# Autodesk Inventor assembly: OpticsTable_Shelf
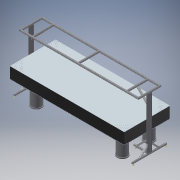
[picture p0: Inventor's stored thumbnail of the model, 180x180]
Saved by Autodesk Inventor 2018 (Build 220112000, 112)
## iProperties
Created: 2018-01-27
Part Number: OpticsTable_Shelf
Document SubType Name: Assembly
Designer: Rich
Author: Rich
## Documents named in this file (14)
- C:\Users\Rich\development\UWaterloo\opticstable_shelf\OpticsTable_Shelf.iam
- C:\Users\Rich\development\UWaterloo\opticstable_shelf\8020-1515-LS-1515-LS X 310cm.ipt
- C:\Users\Rich\development\UWaterloo\opticstable_shelf\8020-1545-S-1545-S X 54.ipt
- C:\Users\Rich\development\UWaterloo\opticstable_shelf\8020-1515-LS-1515-LS X 24.ipt
- C:\Users\Rich\development\UWaterloo\opticstable_shelf\8020-1515-LS-1515-LS X 21.ipt
- C:\Users\Rich\development\UWaterloo\opticstable_shelf\8020 Original Parts\8020-3660-DEFAULT.ipt
- C:\Users\Rich\development\UWaterloo\opticstable_shelf\8020-1515-LS-1515-LS X 36.ipt
- C:\Users\Rich\development\UWaterloo\opticstable_shelf\8020 Original Parts\8020-2561-$PARTNUMBER.ipt
- C:\Users\Rich\development\UWaterloo\opticstable_shelf\8020 Original Parts\8020-2563-$PARTNUMBER.ipt
- C:\Users\Rich\development\UWaterloo\opticstable_shelf\8020 Original Parts\8020-2190-DEFAULT.ipt
- C:\Users\Rich\development\UWaterloo\opticstable_shelf\8020 Original Parts\8020-2200-DEFAULT.ipt
- C:\Users\Rich\development\UWaterloo\opticstable_shelf\8020-1515-S-1515-S X 15.ipt
- C:\Users\Rich\development\UWaterloo\opticstable_shelf\8020 Original Parts\RS2000-410-12.ipt
- C:\Users\Rich\development\UWaterloo\opticstable_shelf\8020 Original Parts\Newport SL 1200-422.ipt
## Components (53 placed, 13 different names)
1. 8020-1545-S-1545-S X 54:1 — Flush:14, Mate:8, Mate:12, Flush:21, Flush:22, Flush:26, Mate:18, Mate:25, Flush:29, Mate:26, Flush:33, Flush:37, Mate:32, Angle:6, Flush:38, Mate:33, Angle:7, Flush:41, Mate:36, Angle:10, Flush:42, Mate:37, Angle:11, Mate:50, Flush:53
2. 8020-1515-LS-1515-LS X 310cm:1 — Mate:3, Flush:5, Flush:6, Flush:11, Mate:6, Flush:12, Mate:9, Flush:15, Mate:10, Flush:16, Flush:24, Mate:13, Flush:25, Mate:14, Angle:1
3. 8020-1515-LS-1515-LS X 310cm:2 — Mate:4, Flush:7, Flush:8, Mate:5, Flush:9, Flush:10, Flush:17, Mate:11, Flush:31, Mate:28, Angle:2, Flush:32, Mate:29, Angle:3
4. 8020-1545-S-1545-S X 54:2 — Mate:2, Flush:4, Mate:7, Flush:13, Flush:18, Flush:20, Flush:21, Mate:15, Mate:16, Mate:21, Flush:27, Mate:23, Flush:34, Mate:30, Flush:35, Angle:4, Mate:31, Flush:36, Angle:5, Flush:39, Mate:34, Angle:8, Flush:40, Mate:35, Angle:9, Mate:49, Flush:52
5. 8020-1515-LS-1515-LS X 24:1 — Mate:5, Flush:9, Flush:10, Flush:11, Mate:6, Flush:12, Flush:14, Mate:8
6. 8020-1515-LS-1515-LS X 24:2 — Mate:3, Flush:5, Flush:6, Mate:4, Flush:7, Flush:8, Mate:7, Flush:13, Flush:20, Flush:23
7. 8020-1515-LS-1515-LS X 21:1 — Mate:9, Flush:15, Mate:17, Mate:46, Flush:51, Angle:16, Mate:47, Mate:48, Angle:17
8. 8020-1515-LS-1515-LS X 21:2 — Mate:10, Flush:16, Flush:23, Mate:44, Flush:49, Angle:14, Mate:45, Flush:50, Angle:15
9. 8020-1515-LS-1515-LS X 21:3 — Flush:17, Mate:11, Mate:19, Flush:47, Mate:42, Angle:12, Flush:48, Mate:43, Angle:13
10. 8020-1515-LS-1515-LS X 36:1 — Mate:12, Flush:19, Flush:22, Mate:24, Mate:27, Flush:30, Mate:38, Flush:43, Mate:39, Flush:44, Mate:51, Flush:54
11. 8020-1515-LS-1515-LS X 36:2 — Mate:1, Mate:2, Flush:4, Flush:18, Flush:19, Mate:20, Mate:22, Flush:28, Mate:40, Flush:45, Mate:41, Flush:46, Mate:52, Flush:56
12. 8020-3660-DEFAULT:1 — Flush:24, Mate:13, Angle:1
13. 8020-3660-DEFAULT:2 — Flush:25, Mate:14
14. 8020-2561-$PARTNUMBER:1 — Mate:22, Mate:23, Flush:28
15. 8020-2561-$PARTNUMBER:2 — Mate:24, Mate:25, Flush:29
16. 8020-2563-$PARTNUMBER:1 — Mate:16, Mate:17, Flush:34
17. 8020-2563-$PARTNUMBER:2 — Mate:18, Mate:19, Flush:33
18. 8020-2561-$PARTNUMBER:3 — Mate:26, Mate:27, Flush:30
19. 8020-2561-$PARTNUMBER:4 — Mate:20, Mate:21, Flush:27
20. 8020-2190-DEFAULT:1
21. 8020-2190-DEFAULT:2
22. 8020-2190-DEFAULT:3
23. 8020-3660-DEFAULT:3 — Flush:31, Mate:28, Angle:2
24. 8020-3660-DEFAULT:4 — Flush:32, Mate:29, Angle:3
25. 8020-3660-DEFAULT:5 — Mate:30, Flush:35, Angle:4
26. 8020-3660-DEFAULT:6 — Mate:31, Flush:36, Angle:5
27. 8020-3660-DEFAULT:7 — Flush:37, Mate:32, Angle:6
28. 8020-3660-DEFAULT:8 — Flush:38, Mate:33, Angle:7
29. 8020-3660-DEFAULT:9 — Flush:39, Mate:34, Angle:8
30. 8020-3660-DEFAULT:10 — Flush:40, Mate:35, Angle:9
31. 8020-3660-DEFAULT:11 — Flush:41, Mate:36, Angle:10
32. 8020-3660-DEFAULT:12 — Flush:42, Mate:37, Angle:11
33. 8020-2200-DEFAULT:1 — Mate:38, Flush:43
34. 8020-2200-DEFAULT:2 — Mate:39, Flush:44
35. 8020-2200-DEFAULT:3 — Mate:40, Flush:45
36. 8020-2200-DEFAULT:4 — Mate:41, Flush:46
37. 8020-3660-DEFAULT:13 — Flush:47, Mate:42, Angle:12
38. 8020-3660-DEFAULT:14 — Flush:48, Mate:43, Angle:13
39. 8020-3660-DEFAULT:15 — Mate:44, Flush:49, Angle:14
40. 8020-3660-DEFAULT:16 — Mate:45, Flush:50, Angle:15
41. 8020-3660-DEFAULT:17 — Mate:46, Flush:51, Angle:16
42. 8020-3660-DEFAULT:18 — Mate:47, Mate:48, Angle:17
43. 8020-2563-$PARTNUMBER:3 — Mate:49, Flush:52, Flush:57, Mate:53
44. 8020-2563-$PARTNUMBER:4 — Mate:50, Flush:53, Flush:55, Mate:54
45. 8020-1515-S-1515-S X 15:1 — Mate:51, Flush:54, Flush:55, Mate:54, Mate:56, Flush:59
46. 8020-1515-S-1515-S X 15:2 — Mate:52, Flush:56, Flush:57, Mate:53, Mate:55, Flush:58
47. 8020-2200-DEFAULT:5 — Mate:55, Flush:58
48. 8020-2200-DEFAULT:6 — Mate:56, Flush:59
49. RS2000-410-12:1 — Mate:57, Mate:58, Flush:60
50. Newport SL 1200-422:1 — Mate:57, Mate:58, Flush:60, Mate:59
51. Newport SL 1200-422:2
52. Newport SL 1200-422:3
53. Newport SL 1200-422:4
## Component patterns: (4 elements, first: Newport SL 1200-422:1)
## Relationships (133: Mate 59, Flush 57, Angle 17)
- Mate:1: 8020-1515-LS-1515-LS X 36:2
- Mate:2: 8020-1545-S-1545-S X 54:2 ↔ 8020-1515-LS-1515-LS X 36:2
- Flush:4: 8020-1545-S-1545-S X 54:2 ↔ 8020-1515-LS-1515-LS X 36:2
- Mate:3: 8020-1515-LS-1515-LS X 310cm:1 ↔ 8020-1515-LS-1515-LS X 24:2
- Flush:5: 8020-1515-LS-1515-LS X 310cm:1 ↔ 8020-1515-LS-1515-LS X 24:2
- Flush:6: 8020-1515-LS-1515-LS X 310cm:1 ↔ 8020-1515-LS-1515-LS X 24:2
- Mate:4: 8020-1515-LS-1515-LS X 310cm:2 ↔ 8020-1515-LS-1515-LS X 24:2
- Flush:7: 8020-1515-LS-1515-LS X 310cm:2 ↔ 8020-1515-LS-1515-LS X 24:2
- Flush:8: 8020-1515-LS-1515-LS X 310cm:2 ↔ 8020-1515-LS-1515-LS X 24:2
- Mate:5: 8020-1515-LS-1515-LS X 310cm:2 ↔ 8020-1515-LS-1515-LS X 24:1
- Flush:9: 8020-1515-LS-1515-LS X 310cm:2 ↔ 8020-1515-LS-1515-LS X 24:1
- Flush:10: 8020-1515-LS-1515-LS X 310cm:2 ↔ 8020-1515-LS-1515-LS X 24:1
- Flush:11: 8020-1515-LS-1515-LS X 310cm:1 ↔ 8020-1515-LS-1515-LS X 24:1
- Mate:6: 8020-1515-LS-1515-LS X 310cm:1 ↔ 8020-1515-LS-1515-LS X 24:1
- Flush:12: 8020-1515-LS-1515-LS X 310cm:1 ↔ 8020-1515-LS-1515-LS X 24:1
- Mate:7: 8020-1545-S-1545-S X 54:2 ↔ 8020-1515-LS-1515-LS X 24:2
- Flush:13: 8020-1545-S-1545-S X 54:2 ↔ 8020-1515-LS-1515-LS X 24:2
- Flush:14: 8020-1545-S-1545-S X 54:1 ↔ 8020-1515-LS-1515-LS X 24:1
- Mate:8: 8020-1545-S-1545-S X 54:1 ↔ 8020-1515-LS-1515-LS X 24:1
- Mate:9: 8020-1515-LS-1515-LS X 310cm:1 ↔ 8020-1515-LS-1515-LS X 21:1
- Flush:15: 8020-1515-LS-1515-LS X 310cm:1 ↔ 8020-1515-LS-1515-LS X 21:1
- Mate:10: 8020-1515-LS-1515-LS X 310cm:1 ↔ 8020-1515-LS-1515-LS X 21:2
- Flush:16: 8020-1515-LS-1515-LS X 310cm:1 ↔ 8020-1515-LS-1515-LS X 21:2
- Flush:17: 8020-1515-LS-1515-LS X 310cm:2 ↔ 8020-1515-LS-1515-LS X 21:3
- Mate:11: 8020-1515-LS-1515-LS X 310cm:2 ↔ 8020-1515-LS-1515-LS X 21:3
- Mate:12: 8020-1545-S-1545-S X 54:1 ↔ 8020-1515-LS-1515-LS X 36:1
- Flush:18 (-400.05 mm): 8020-1545-S-1545-S X 54:2 ↔ 8020-1515-LS-1515-LS X 36:2
- Flush:19: 8020-1515-LS-1515-LS X 36:1 ↔ 8020-1515-LS-1515-LS X 36:2
- Flush:20 (247.65 mm): 8020-1545-S-1545-S X 54:2 ↔ 8020-1515-LS-1515-LS X 24:2
- Flush:21: 8020-1545-S-1545-S X 54:1 ↔ 8020-1545-S-1545-S X 54:2
- Flush:22: 8020-1545-S-1545-S X 54:1 ↔ 8020-1515-LS-1515-LS X 36:1
- Flush:23 (-1530.95 mm): 8020-1515-LS-1515-LS X 24:2 ↔ 8020-1515-LS-1515-LS X 21:2
- Flush:24: 8020-1515-LS-1515-LS X 310cm:1 ↔ 8020-3660-DEFAULT:1
- Mate:13: 8020-1515-LS-1515-LS X 310cm:1 ↔ 8020-3660-DEFAULT:1
- Flush:25: 8020-1515-LS-1515-LS X 310cm:1 ↔ 8020-3660-DEFAULT:2
- Mate:14: 8020-1515-LS-1515-LS X 310cm:1 ↔ 8020-3660-DEFAULT:2
- Flush:26: 8020-1545-S-1545-S X 54:1
- Angle:1 (0 deg): 8020-1515-LS-1515-LS X 310cm:1 ↔ 8020-3660-DEFAULT:1
- Mate:15: 8020-1545-S-1545-S X 54:2
- Mate:16: 8020-1545-S-1545-S X 54:2 ↔ 8020-2563-$PARTNUMBER:1
- Mate:17: 8020-1515-LS-1515-LS X 21:1 ↔ 8020-2563-$PARTNUMBER:1
- Mate:18: 8020-1545-S-1545-S X 54:1 ↔ 8020-2563-$PARTNUMBER:2
- Mate:19: 8020-1515-LS-1515-LS X 21:3 ↔ 8020-2563-$PARTNUMBER:2
- Mate:20: 8020-1515-LS-1515-LS X 36:2 ↔ 8020-2561-$PARTNUMBER:4
- Mate:21: 8020-1545-S-1545-S X 54:2 ↔ 8020-2561-$PARTNUMBER:4
- Flush:27: 8020-1545-S-1545-S X 54:2 ↔ 8020-2561-$PARTNUMBER:4
- Mate:22: 8020-1515-LS-1515-LS X 36:2 ↔ 8020-2561-$PARTNUMBER:1
- Mate:23: 8020-1545-S-1545-S X 54:2 ↔ 8020-2561-$PARTNUMBER:1
- Flush:28: 8020-1515-LS-1515-LS X 36:2 ↔ 8020-2561-$PARTNUMBER:1
- Mate:24: 8020-1515-LS-1515-LS X 36:1 ↔ 8020-2561-$PARTNUMBER:2
- Mate:25: 8020-1545-S-1545-S X 54:1 ↔ 8020-2561-$PARTNUMBER:2
- Flush:29: 8020-1545-S-1545-S X 54:1 ↔ 8020-2561-$PARTNUMBER:2
- Mate:26: 8020-1545-S-1545-S X 54:1 ↔ 8020-2561-$PARTNUMBER:3
- Mate:27: 8020-1515-LS-1515-LS X 36:1 ↔ 8020-2561-$PARTNUMBER:3
- Flush:30: 8020-1515-LS-1515-LS X 36:1 ↔ 8020-2561-$PARTNUMBER:3
- Flush:31: 8020-1515-LS-1515-LS X 310cm:2 ↔ 8020-3660-DEFAULT:3
- Mate:28: 8020-1515-LS-1515-LS X 310cm:2 ↔ 8020-3660-DEFAULT:3
- Angle:2 (180 deg): 8020-1515-LS-1515-LS X 310cm:2 ↔ 8020-3660-DEFAULT:3
- Flush:32: 8020-1515-LS-1515-LS X 310cm:2 ↔ 8020-3660-DEFAULT:4
- Mate:29: 8020-1515-LS-1515-LS X 310cm:2 ↔ 8020-3660-DEFAULT:4
- Angle:3 (180 deg): 8020-1515-LS-1515-LS X 310cm:2 ↔ 8020-3660-DEFAULT:4
- Flush:33 (38.1 mm): 8020-1545-S-1545-S X 54:1 ↔ 8020-2563-$PARTNUMBER:2
- Flush:34 (-38.1 mm): 8020-1545-S-1545-S X 54:2 ↔ 8020-2563-$PARTNUMBER:1
- Mate:30: 8020-1545-S-1545-S X 54:2 ↔ 8020-3660-DEFAULT:5
- Flush:35: 8020-1545-S-1545-S X 54:2 ↔ 8020-3660-DEFAULT:5
- Angle:4 (180 deg): 8020-1545-S-1545-S X 54:2 ↔ 8020-3660-DEFAULT:5
- Mate:31: 8020-1545-S-1545-S X 54:2 ↔ 8020-3660-DEFAULT:6
- Flush:36: 8020-1545-S-1545-S X 54:2 ↔ 8020-3660-DEFAULT:6
- Angle:5 (180 deg): 8020-1545-S-1545-S X 54:2 ↔ 8020-3660-DEFAULT:6
- Flush:37: 8020-1545-S-1545-S X 54:1 ↔ 8020-3660-DEFAULT:7
- Mate:32: 8020-1545-S-1545-S X 54:1 ↔ 8020-3660-DEFAULT:7
- Angle:6 (180 deg): 8020-1545-S-1545-S X 54:1 ↔ 8020-3660-DEFAULT:7
- Flush:38: 8020-1545-S-1545-S X 54:1 ↔ 8020-3660-DEFAULT:8
- Mate:33: 8020-1545-S-1545-S X 54:1 ↔ 8020-3660-DEFAULT:8
- Angle:7 (0 deg): 8020-1545-S-1545-S X 54:1 ↔ 8020-3660-DEFAULT:8
- Flush:39: 8020-1545-S-1545-S X 54:2 ↔ 8020-3660-DEFAULT:9
- Mate:34: 8020-1545-S-1545-S X 54:2 ↔ 8020-3660-DEFAULT:9
- Angle:8 (0 deg): 8020-1545-S-1545-S X 54:2 ↔ 8020-3660-DEFAULT:9
- Flush:40: 8020-1545-S-1545-S X 54:2 ↔ 8020-3660-DEFAULT:10
- Mate:35: 8020-1545-S-1545-S X 54:2 ↔ 8020-3660-DEFAULT:10
- Angle:9 (0 deg): 8020-1545-S-1545-S X 54:2 ↔ 8020-3660-DEFAULT:10
- Flush:41: 8020-1545-S-1545-S X 54:1 ↔ 8020-3660-DEFAULT:11
- Mate:36: 8020-1545-S-1545-S X 54:1 ↔ 8020-3660-DEFAULT:11
- Angle:10 (180 deg): 8020-1545-S-1545-S X 54:1 ↔ 8020-3660-DEFAULT:11
- Flush:42: 8020-1545-S-1545-S X 54:1 ↔ 8020-3660-DEFAULT:12
- Mate:37: 8020-1545-S-1545-S X 54:1 ↔ 8020-3660-DEFAULT:12
- Angle:11 (180 deg): 8020-1545-S-1545-S X 54:1 ↔ 8020-3660-DEFAULT:12
- Mate:38: 8020-1515-LS-1515-LS X 36:1 ↔ 8020-2200-DEFAULT:1
- Flush:43 (-38.1 mm): 8020-1515-LS-1515-LS X 36:1 ↔ 8020-2200-DEFAULT:1
- Mate:39: 8020-1515-LS-1515-LS X 36:1 ↔ 8020-2200-DEFAULT:2
- Flush:44 (38.1 mm): 8020-1515-LS-1515-LS X 36:1 ↔ 8020-2200-DEFAULT:2
- Mate:40: 8020-1515-LS-1515-LS X 36:2 ↔ 8020-2200-DEFAULT:3
- Flush:45 (38.1 mm): 8020-1515-LS-1515-LS X 36:2 ↔ 8020-2200-DEFAULT:3
- Mate:41: 8020-1515-LS-1515-LS X 36:2 ↔ 8020-2200-DEFAULT:4
- Flush:46 (38.1 mm): 8020-1515-LS-1515-LS X 36:2 ↔ 8020-2200-DEFAULT:4
- Flush:47: 8020-1515-LS-1515-LS X 21:3 ↔ 8020-3660-DEFAULT:13
- Mate:42: 8020-1515-LS-1515-LS X 21:3 ↔ 8020-3660-DEFAULT:13
- Angle:12 (0 deg): 8020-1515-LS-1515-LS X 21:3 ↔ 8020-3660-DEFAULT:13
- Flush:48: 8020-1515-LS-1515-LS X 21:3 ↔ 8020-3660-DEFAULT:14
- Mate:43: 8020-1515-LS-1515-LS X 21:3 ↔ 8020-3660-DEFAULT:14
- Angle:13 (180 deg): 8020-1515-LS-1515-LS X 21:3 ↔ 8020-3660-DEFAULT:14
- Mate:44: 8020-1515-LS-1515-LS X 21:2 ↔ 8020-3660-DEFAULT:15
- Flush:49: 8020-1515-LS-1515-LS X 21:2 ↔ 8020-3660-DEFAULT:15
- Angle:14 (0 deg): 8020-1515-LS-1515-LS X 21:2 ↔ 8020-3660-DEFAULT:15
- Mate:45: 8020-1515-LS-1515-LS X 21:2 ↔ 8020-3660-DEFAULT:16
- Flush:50: 8020-1515-LS-1515-LS X 21:2 ↔ 8020-3660-DEFAULT:16
- Angle:15 (180 deg): 8020-1515-LS-1515-LS X 21:2 ↔ 8020-3660-DEFAULT:16
- Mate:46: 8020-1515-LS-1515-LS X 21:1 ↔ 8020-3660-DEFAULT:17
- Flush:51: 8020-1515-LS-1515-LS X 21:1 ↔ 8020-3660-DEFAULT:17
- Angle:16 (0 deg): 8020-1515-LS-1515-LS X 21:1 ↔ 8020-3660-DEFAULT:17
- Mate:47: 8020-1515-LS-1515-LS X 21:1 ↔ 8020-3660-DEFAULT:18
- Mate:48: 8020-1515-LS-1515-LS X 21:1 ↔ 8020-3660-DEFAULT:18
- Angle:17 (180 deg): 8020-1515-LS-1515-LS X 21:1 ↔ 8020-3660-DEFAULT:18
- Mate:49: 8020-1545-S-1545-S X 54:2 ↔ 8020-2563-$PARTNUMBER:3
- Flush:52 (38.1 mm): 8020-1545-S-1545-S X 54:2 ↔ 8020-2563-$PARTNUMBER:3
- Mate:50: 8020-1545-S-1545-S X 54:1 ↔ 8020-2563-$PARTNUMBER:4
- Flush:53 (38.1 mm): 8020-1545-S-1545-S X 54:1 ↔ 8020-2563-$PARTNUMBER:4
- Mate:51: 8020-1515-LS-1515-LS X 36:1 ↔ 8020-1515-S-1515-S X 15:1
- Flush:54: 8020-1515-LS-1515-LS X 36:1 ↔ 8020-1515-S-1515-S X 15:1
- Flush:55: 8020-2563-$PARTNUMBER:4 ↔ 8020-1515-S-1515-S X 15:1
- Mate:52: 8020-1515-LS-1515-LS X 36:2 ↔ 8020-1515-S-1515-S X 15:2
- Flush:56: 8020-1515-LS-1515-LS X 36:2 ↔ 8020-1515-S-1515-S X 15:2
- Flush:57: 8020-2563-$PARTNUMBER:3 ↔ 8020-1515-S-1515-S X 15:2
- Mate:53: 8020-2563-$PARTNUMBER:3 ↔ 8020-1515-S-1515-S X 15:2
- Mate:54: 8020-2563-$PARTNUMBER:4 ↔ 8020-1515-S-1515-S X 15:1
- Mate:55: 8020-1515-S-1515-S X 15:2 ↔ 8020-2200-DEFAULT:5
- Flush:58 (-38.1 mm): 8020-1515-S-1515-S X 15:2 ↔ 8020-2200-DEFAULT:5
- Mate:56: 8020-1515-S-1515-S X 15:1 ↔ 8020-2200-DEFAULT:6
- Flush:59 (38.1 mm): 8020-1515-S-1515-S X 15:1 ↔ 8020-2200-DEFAULT:6
- Mate:57: RS2000-410-12:1 ↔ Newport SL 1200-422:1
- Mate:58 (-457.2 mm): RS2000-410-12:1 ↔ Newport SL 1200-422:1
- Flush:60 (254 mm): RS2000-410-12:1 ↔ Newport SL 1200-422:1
- Mate:59: Newport SL 1200-422:1
